# Autodesk Inventor assembly: main
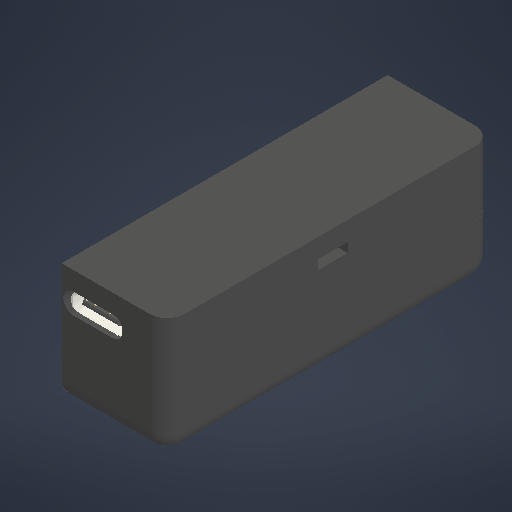
[picture p0: Inventor's stored thumbnail of the model, 512x512]
Saved by Autodesk Inventor 2026.2 (Build 302298000, 298)
## iProperties
Created: 2025-12-22
Part Number: main
Document SubType Name: Assembly
Designer: test
Author: test
## Documents named in this file (6)
- C:\Users\test\Projects\WearableWLED\WearableWLED_Mechanical\main.iam
- C:\Users\test\Projects\WearableWLED\WearableWLED_Mechanical\case1.ipt
- C:\Users\test\Projects\WearableWLED\WearableWLED_Mechanical\battery.ipt
- C:\Users\test\Projects\WearableWLED\WearableWLED_Mechanical\case2.ipt
- C:\Users\test\Projects\WearableWLED\WearableWLED_Mechanical\board\WearableWLED_Hardware\WearableWLED_Hardware\WearableWLED_Hardware.iam
- C:\Users\test\Projects\WearableWLED\WearableWLED_Mechanical\dimmensions.xlsx
## Components (4 placed, 4 different names)
1. case1:1 — Zestawiające:2, Zestawiające:3, Zestawiające:4, Równoległe:1, Równoległe:2, Zestawiające:8
2. battery:1 — Zestawiające:2, Zestawiające:3, Zestawiające:4
3. case2:1 — Równoległe:1, Równoległe:2, Zestawiające:5, Zestawiające:6, Zestawiające:7, Zestawiające:8
4. WearableWLED_Hardware:1 [sub-assembly] — Zestawiające:5, Zestawiające:6, Zestawiające:7
## Relationships (9: Mate 7, Flush 2)
- Zestawiające:2 [Mate]: case1:1 ↔ battery:1
- Zestawiające:3 [Mate]: case1:1 ↔ battery:1
- Zestawiające:4 [Mate]: case1:1 ↔ battery:1
- Równoległe:1 [Flush]: case1:1 ↔ case2:1
- Równoległe:2 [Flush]: case1:1 ↔ case2:1
- Zestawiające:5 [Mate] (0.5 mm): case2:1 ↔ WearableWLED_Hardware:1
- Zestawiające:6 [Mate]: case2:1 ↔ WearableWLED_Hardware:1
- Zestawiające:7 [Mate]: case2:1 ↔ WearableWLED_Hardware:1
- Zestawiające:8 [Mate]: case1:1 ↔ case2:1
## Named parameters: wall_thickness = 2 mm, case_h = 16 mm, case_d = 51 mm, case_w = 21 mm, case_ratio = 0.5, case_mounting = 0.8 mm
note: some values were not read from the file. Shown as the stored number, unit unknown: "case_ratio".
